# Autodesk Inventor assembly: hingeee
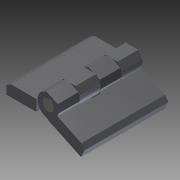
[picture p0: Inventor's stored thumbnail of the model, 180x180]
Saved by Autodesk Inventor 2015 (Build 190159000, 159)
## iProperties
Created: 2015-07-08
Part Number: hingeee
Document SubType Name: Assembly
Designer: Owner
Author: Owner
## Documents named in this file (4)
- C:\Users\Owner\Documents\GrabCAD\Driver Station\hingeee.iam
- C:\Users\Owner\Documents\GrabCAD\Driver Station\Imported Components\hinge1\Part2.ipt
- C:\Users\Owner\Documents\GrabCAD\Driver Station\Imported Components\hinge1\Part4.ipt
- C:\Users\Owner\Documents\GrabCAD\Driver Station\Imported Components\hinge1\Part6.ipt
## Components (3 placed, 3 different names)
1. Part2:1 — Mate:2, Flush:2
2. Part4:1 — Mate:1, Flush:1, Flush:2
3. Part6:1 — Mate:1, Mate:2, Flush:1
## Relationships (4: Mate 2, Flush 2)
- Mate:1: Part4:1 ↔ Part6:1
- Mate:2: Part2:1 ↔ Part6:1
- Flush:1: Part4:1 ↔ Part6:1
- Flush:2: Part2:1 ↔ Part4:1
